# Autodesk Inventor assembly: Assembly1
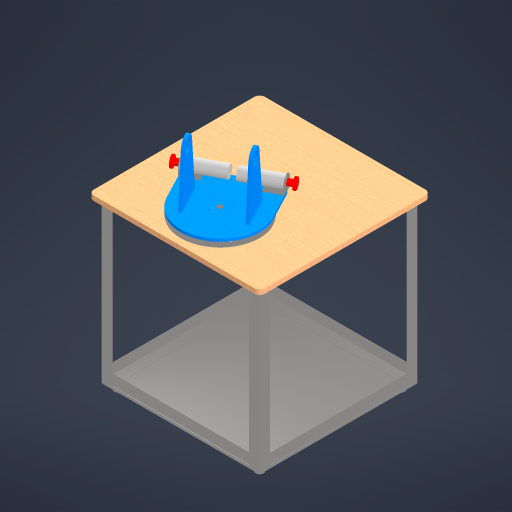
[picture p0: Inventor's stored thumbnail of the model, 512x512]
Saved by Autodesk Inventor 2023 (Build 270158000, 158)
## iProperties
Created: 2023-09-08
Part Number: Assembly1
Document SubType Name: Assembly
Designer: Abhinav
Author: Abhinav
## Documents named in this file (13)
- C:\Users\Abhinav\Desktop\GRID\ARM 3\Foundation\00_Foundation.iam
- C:\Users\Abhinav\Desktop\GRID\ARM 3\Foundation\Foundation-Fork.ipt
- C:\Users\Abhinav\Desktop\GRID\ARM 3\Foundation\Castor.ipt
- C:\Users\Abhinav\Desktop\GRID\ARM 3\Foundation\DC Motor 100kgcm.ipt
- C:\Users\Abhinav\Desktop\GRID\ARM 3\Foundation\Foundation-Base.ipt
- C:\Users\Abhinav\Desktop\GRID\ARM 3\Foundation\Compressor.ipt
- C:\Users\Abhinav\Desktop\GRID\ARM 3\Foundation\Base_Motor_Mount.ipt
- C:\Users\Abhinav\Desktop\GRID\ARM 3\Foundation\Bearing Plate.ipt
- C:\Users\Abhinav\Desktop\GRID\ARM 3\Foundation\Foundation-Motor-Mount.ipt
- C:\Users\Abhinav\Desktop\GRID\ARM 3\Foundation\Roller-Plate.ipt
- C:\Users\Abhinav\Desktop\GRID\ARM 3\Foundation\11T-Sprocket.ipt
- C:\Users\Abhinav\Desktop\GRID\ARM 3\Foundation\56T-Sprocket.ipt
- C:\Users\Abhinav\Desktop\GRID\ARM 3\Foundation\Base-Shaft.ipt
## Components (22 placed, 12 different names)
1. Foundation-Fork:1 — Mate:1, Mate:2, Mate:3, Mate:4, Mate:5, Mate:6, Mate:7, Mate:8, Mate:9, Mate:10, Mate:11, Mate:12, Mate:15, Mate:16, Mate:17, Mate:18, Mate:19, Mate:20, Angle:1, Mate:22, Mate:39, Mate:40, Flush:4, Flush:5, Flush:6, Flush:7, Flush:51, Mate:50
2. Castor:1 — Mate:4, Mate:11, Mate:12
3. Castor:2 — Mate:2, Mate:7, Mate:8
4. Castor:3 — Mate:3, Mate:9, Mate:10
5. Castor:4 — Mate:1, Mate:5, Mate:6
6. Castor:5 — Mate:15, Mate:19, Mate:20
7. Castor:6 — Mate:16, Mate:17, Mate:18, Tangent:1
8. Foundation-Base:1 — Mate:21, Mate:22, Mate:25, Flush:3, Mate:26, Mate:27, Mate:28, Bear_Plate_1, Bear_Plate_2, Mate:41
9. Compressor:1 — Mate:25, Flush:3
10. Base_Motor_Mount:1 — Mate:26, Mate:27, Mate:28, Mate:29, Mate:30, Mate:31, Mate:48
11. DC Motor 100kgcm:3 — Mate:29, Mate:30, Mate:31, Mate:47
12. Bearing Plate:1 — Bear_Plate, Bear_Plate_1, Bear_Plate_2, Mate:42
13. Foundation-Motor-Mount:1 — Mate:36, Mate:37, Mate:39, Flush:4, Flush:6, Sp-4
14. Foundation-Motor-Mount:2 — Mate:35, Mate:38, Mate:40, Flush:5, Flush:7, Sp-2
15. DC Motor 100kgcm:4 — Mate:36, Mate:37, Sp-3
16. DC Motor 100kgcm:5 — Mate:35, Mate:38, Sp-1
17. Roller-Plate:1 — Bear_Plate, Mate:41, Mate:42
18. 11T-Sprocket:1 — Sp-1, Sp-2
19. 11T-Sprocket:2 — Sp-3, Sp-4
20. 11T-Sprocket:3 — Mate:47, Mate:48, Flush:8
21. 56T-Sprocket:1 — Mate:49, Flush:8
22. Base-Shaft:1 — Flush:51, Mate:50, Mate:49
## Relationships (55: Mate 46, Flush 7, Angle 1, Tangent 1)
- Mate:1: Foundation-Fork:1 ↔ Castor:4
- Mate:2: Foundation-Fork:1 ↔ Castor:2
- Mate:3: Foundation-Fork:1 ↔ Castor:3
- Mate:4: Foundation-Fork:1 ↔ Castor:1
- Mate:5: Foundation-Fork:1 ↔ Castor:4
- Mate:6: Foundation-Fork:1 ↔ Castor:4
- Mate:7: Foundation-Fork:1 ↔ Castor:2
- Mate:8: Foundation-Fork:1 ↔ Castor:2
- Mate:9: Foundation-Fork:1 ↔ Castor:3
- Mate:10: Foundation-Fork:1 ↔ Castor:3
- Mate:11: Foundation-Fork:1 ↔ Castor:1
- Mate:12: Foundation-Fork:1 ↔ Castor:1
- Mate:15: Foundation-Fork:1 ↔ Castor:5
- Mate:16: Foundation-Fork:1 ↔ Castor:6
- Mate:17: Foundation-Fork:1 ↔ Castor:6
- Mate:18: Foundation-Fork:1 ↔ Castor:6
- Mate:19: Foundation-Fork:1 ↔ Castor:5
- Mate:20: Foundation-Fork:1 ↔ Castor:5
- Angle:1 (0 deg): Foundation-Fork:1
- Tangent:1: Castor:6
- Mate:21: Foundation-Base:1
- Mate:22: Foundation-Fork:1 ↔ Foundation-Base:1
- Mate:25: Foundation-Base:1 ↔ Compressor:1
- Flush:3: Foundation-Base:1 ↔ Compressor:1
- Mate:26: Foundation-Base:1 ↔ Base_Motor_Mount:1
- Mate:27: Foundation-Base:1 ↔ Base_Motor_Mount:1
- Mate:28: Foundation-Base:1 ↔ Base_Motor_Mount:1
- Mate:29: Base_Motor_Mount:1 ↔ DC Motor 100kgcm:3
- Mate:30: Base_Motor_Mount:1 ↔ DC Motor 100kgcm:3
- Mate:31: Base_Motor_Mount:1 ↔ DC Motor 100kgcm:3
- Bear_Plate [Mate]: Bearing Plate:1 ↔ Roller-Plate:1
- Bear_Plate_1 [Mate]: Foundation-Base:1 ↔ Bearing Plate:1
- Bear_Plate_2 [Mate]: Foundation-Base:1 ↔ Bearing Plate:1
- Mate:35: Foundation-Motor-Mount:2 ↔ DC Motor 100kgcm:5
- Mate:36: Foundation-Motor-Mount:1 ↔ DC Motor 100kgcm:4
- Mate:37: Foundation-Motor-Mount:1 ↔ DC Motor 100kgcm:4
- Mate:38: Foundation-Motor-Mount:2 ↔ DC Motor 100kgcm:5
- Mate:39: Foundation-Fork:1 ↔ Foundation-Motor-Mount:1
- Mate:40: Foundation-Fork:1 ↔ Foundation-Motor-Mount:2
- Flush:4: Foundation-Fork:1 ↔ Foundation-Motor-Mount:1
- Flush:5: Foundation-Fork:1 ↔ Foundation-Motor-Mount:2
- Flush:6: Foundation-Fork:1 ↔ Foundation-Motor-Mount:1
- Flush:7: Foundation-Fork:1 ↔ Foundation-Motor-Mount:2
- Mate:41: Foundation-Base:1 ↔ Roller-Plate:1
- Mate:42: Bearing Plate:1 ↔ Roller-Plate:1
- Sp-1 [Mate]: DC Motor 100kgcm:5 ↔ 11T-Sprocket:1
- Sp-2 [Mate]: Foundation-Motor-Mount:2 ↔ 11T-Sprocket:1
- Sp-3 [Mate]: DC Motor 100kgcm:4 ↔ 11T-Sprocket:2
- Sp-4 [Mate]: Foundation-Motor-Mount:1 ↔ 11T-Sprocket:2
- Mate:47: DC Motor 100kgcm:3 ↔ 11T-Sprocket:3
- Mate:48: Base_Motor_Mount:1 ↔ 11T-Sprocket:3
- Mate:49: 56T-Sprocket:1 ↔ Base-Shaft:1
- Flush:8: 11T-Sprocket:3 ↔ 56T-Sprocket:1
- Flush:51: Foundation-Fork:1 ↔ Base-Shaft:1
- Mate:50: Foundation-Fork:1 ↔ Base-Shaft:1
